# Autodesk Inventor assembly: Printhead
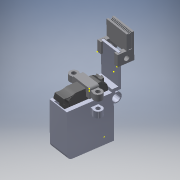
[picture p0: Inventor's stored thumbnail of the model, 180x180]
Saved by Autodesk Inventor 2018 (Build 220112000, 112)
## iProperties
Created: 2018-03-15
Part Number: Printhead
Document SubType Name: Assembly
Designer: junai
Author: junai
## Documents named in this file (5)
- C:\Users\junai\Documents\Sensors\pH Free Cl Sensor\DIY_Inkjet_Printer\Mechanical\Printhead.iam
- C:\Users\junai\Documents\Sensors\pH Free Cl Sensor\DIY_Inkjet_Printer\Mechanical\HP45.ipt
- C:\Users\junai\Documents\Sensors\pH Free Cl Sensor\DIY_Inkjet_Printer\Mechanical\HP45 Printhead Cap.ipt
- C:\Users\junai\Documents\Sensors\pH Free Cl Sensor\DIY_Inkjet_Printer\Mechanical\HP45 Printhead Holder.ipt
- C:\Users\junai\Documents\Sensors\pH Free Cl Sensor\DIY_Inkjet_Printer\Mechanical\Y Belt Holder.ipt
## Components (4 placed, 4 different names)
1. HP45:1
2. HP45 Printhead Cap:1 — Mate:1, Mate:2
3. HP45 Printhead Holder:1 — Mate:1, Mate:2, Flush:1, Flush:2
4. Y Belt Holder:1 — Flush:1, Flush:2
## Relationships (4: Mate 2, Flush 2)
- Mate:1: HP45 Printhead Cap:1 ↔ HP45 Printhead Holder:1
- Mate:2: HP45 Printhead Cap:1 ↔ HP45 Printhead Holder:1
- Flush:1: HP45 Printhead Holder:1 ↔ Y Belt Holder:1
- Flush:2: HP45 Printhead Holder:1 ↔ Y Belt Holder:1
